# Autodesk Inventor assembly: Wheel Orientation
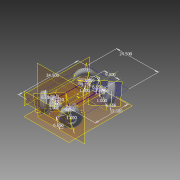
[picture p0: Inventor's stored thumbnail of the model, 180x180]
Saved by Autodesk Inventor 2015 (Build 190159000, 159)
## iProperties
Created: 2016-01-19
Part Number: Wheel Orientation
Document SubType Name: Assembly
Designer: sethbattis
Author: sethbattis
## Documents named in this file (3)
- \\area51\team3566\cad\FRC 2016\Wheel Orientation.iam
- \\area51\team3566\cad\FRC 2016\Wheelbase.ipt
- \\area51\team3566\cad\FRC 2016\Snow Tire Wheel with Gearbox and CIM.ipt
## Components (5 placed, 2 different names)
1. Wheelbase:1 — Rotational:1, Rotational:2, Rotational:3, Rotational:4
2. Snow Tire Wheel with Gearbox and CIM:1 — Rotational:2
3. Snow Tire Wheel with Gearbox and CIM:2 — Rotational:1
4. Snow Tire Wheel with Gearbox and CIM:3 — Rotational:4
5. Snow Tire Wheel with Gearbox and CIM:4 — Rotational:3
## Relationships (5: RevoluteJoint 4, Flush 1)
- Rotational:1 [RevoluteJoint]: Wheelbase:1 ↔ Snow Tire Wheel with Gearbox and CIM:2
- Rotational:2 [RevoluteJoint]: Wheelbase:1 ↔ Snow Tire Wheel with Gearbox and CIM:1
- Rotational:3 [RevoluteJoint]: Wheelbase:1 ↔ Snow Tire Wheel with Gearbox and CIM:4
- Rotational:4 [RevoluteJoint]: Wheelbase:1 ↔ Snow Tire Wheel with Gearbox and CIM:3
- Flush:1 (-169.0624 mm)
